# Autodesk Inventor assembly: Rührreaktor
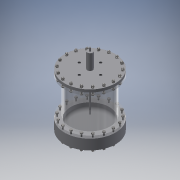
[picture p0: Inventor's stored thumbnail of the model, 180x180]
Saved by Autodesk Inventor 2017 (Build 210142000, 142)
## iProperties
Created: 2019-06-21
Part Number: Rührreaktor
Document SubType Name: Assembly
Designer: Ole Simmering
Author: Ole Simmering
## Documents named in this file (11)
- C:\Users\Ole Simmering\Documents\3d modelling fun\HA5-Rührreaktor\Rührreaktor.iam
- C:\Users\Ole Simmering\Documents\3d modelling fun\HA5-Rührreaktor\Deckelplatte.ipt
- C:\Users\Ole Simmering\Documents\3d modelling fun\HA5-Rührreaktor\Reaktor.ipt
- C:\Users\Ole Simmering\Documents\3d modelling fun\HA5-Rührreaktor\Steckhülse.ipt
- C:\Users\Ole Simmering\Documents\3d modelling fun\HA5-Rührreaktor\Korbbogenboden.ipt
- C:\Users\Ole Simmering\Documents\3d modelling fun\HA5-Rührreaktor\Lagertopf.ipt
- C:\Users\Ole Simmering\Documents\Inventor\Content Center Files\R2017\en-US\DIN 628 SKF(4)\DIN 628 SKF - SKF 7201 BEP.ipt
- C:\Users\Ole Simmering\Documents\3d modelling fun\HA5-Rührreaktor\LagerDeckel.ipt
- C:\Users\Ole Simmering\Documents\3d modelling fun\HA5-Rührreaktor\Achse.ipt
- C:\Users\Ole Simmering\Documents\3d modelling fun\HA5-Rührreaktor\Rührreaktor\Design Accelerator\Bolted Connection2.iam
- C:\Users\Ole Simmering\Documents\3d modelling fun\HA5-Rührreaktor\Rührreaktor\Design Accelerator\Bolted Connection3.iam
## Components (45 placed, 9 different names)
1. Deckelplatte:1 — Mate:1, Mate:2, Cylindrical:1, Mate:7, Mate:13
2. Reaktor:1 — Mate:1, Mate:2, Mate:3, Mate:4, Mate:5, Mate:12, Mate:14
3. Steckhülse:1 — Insert:3, Mate:11
4. Korbbogenboden:1 — Mate:3, Mate:4, Mate:5, Mate:15
5. Lagertopf:1 — Cylindrical:1, Mate:6, Mate:7, Mate:8, Mate:9, Insert:1
6. DIN 628 SKF - 7..B SKF 7201 BEP:1 — Mate:6, Mate:8, Insert:2
7. DIN 628 SKF - 7..B SKF 7201 BEP:2 — Mate:9, Mate:10
8. LagerDeckel:1 — Insert:1, Mate:10
9. Achse:1 — Insert:2, Insert:3, Mate:11
10. Bolted Connection:1 [sub-assembly] — Mate:12, Mate:13
11. Bolted Connection:2 [sub-assembly]
12. Bolted Connection:3 [sub-assembly]
13. Bolted Connection:4 [sub-assembly]
14. Bolted Connection:5 [sub-assembly]
15. Bolted Connection:6 [sub-assembly]
16. Bolted Connection:7 [sub-assembly]
17. Bolted Connection:8 [sub-assembly]
18. Bolted Connection:9 [sub-assembly]
19. Bolted Connection:10 [sub-assembly]
20. Bolted Connection:11 [sub-assembly]
21. Bolted Connection:12 [sub-assembly]
22. Bolted Connection:13 [sub-assembly]
23. Bolted Connection:14 [sub-assembly]
24. Bolted Connection:15 [sub-assembly]
25. Bolted Connection:16 [sub-assembly]
26. Bolted Connection:17 [sub-assembly]
27. Bolted Connection:18 [sub-assembly]
28. Bolted Connection:19 [sub-assembly] — Mate:14, Mate:15
29. Bolted Connection:20 [sub-assembly]
30. Bolted Connection:21 [sub-assembly]
31. Bolted Connection:22 [sub-assembly]
32. Bolted Connection:23 [sub-assembly]
33. Bolted Connection:24 [sub-assembly]
34. Bolted Connection:25 [sub-assembly]
35. Bolted Connection:26 [sub-assembly]
36. Bolted Connection:27 [sub-assembly]
37. Bolted Connection:28 [sub-assembly]
38. Bolted Connection:29 [sub-assembly]
39. Bolted Connection:30 [sub-assembly]
40. Bolted Connection:31 [sub-assembly]
41. Bolted Connection:32 [sub-assembly]
42. Bolted Connection:33 [sub-assembly]
43. Bolted Connection:34 [sub-assembly]
44. Bolted Connection:35 [sub-assembly]
45. Bolted Connection:36 [sub-assembly]
## Component patterns: (18 elements, first: Bolted Connection:1), (18 elements, first: Bolted Connection:19)
## Relationships (19: Mate 15, Insert 3, CylindricalJoint 1)
- Mate:1: Deckelplatte:1 ↔ Reaktor:1
- Mate:2: Deckelplatte:1 ↔ Reaktor:1
- Mate:3: Reaktor:1 ↔ Korbbogenboden:1
- Mate:4: Reaktor:1 ↔ Korbbogenboden:1
- Mate:5: Reaktor:1 ↔ Korbbogenboden:1
- Cylindrical:1: Deckelplatte:1 ↔ Lagertopf:1
- Mate:6: Lagertopf:1 ↔ DIN 628 SKF - 7..B SKF 7201 BEP:1
- Mate:7: Deckelplatte:1 ↔ Lagertopf:1
- Mate:8: Lagertopf:1 ↔ DIN 628 SKF - 7..B SKF 7201 BEP:1
- Mate:9: Lagertopf:1 ↔ DIN 628 SKF - 7..B SKF 7201 BEP:2
- Insert:1 (-10 mm): Lagertopf:1 ↔ LagerDeckel:1
- Insert:2: DIN 628 SKF - 7..B SKF 7201 BEP:1 ↔ Achse:1
- Mate:10: DIN 628 SKF - 7..B SKF 7201 BEP:2 ↔ LagerDeckel:1
- Insert:3: Steckhülse:1 ↔ Achse:1
- Mate:11: Steckhülse:1 ↔ Achse:1
- Mate:12: Reaktor:1 ↔ Bolted Connection:1
- Mate:13: Deckelplatte:1 ↔ Bolted Connection:1
- Mate:14: Reaktor:1 ↔ Bolted Connection:19
- Mate:15: Korbbogenboden:1 ↔ Bolted Connection:19
